# Autodesk Inventor assembly: roller
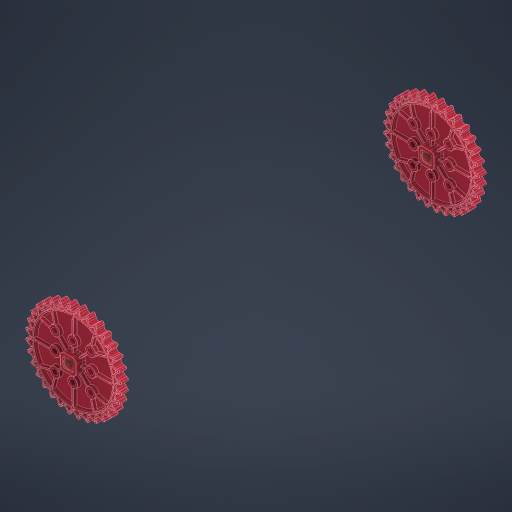
[picture p0: Inventor's stored thumbnail of the model, 512x512]
Saved by Autodesk Inventor 2024 (Build 280153000, 153)
## iProperties
Created: 2023-10-22
Part Number: roller
Document SubType Name: Assembly
Designer: Averey Ku
Author: Averey Ku
## Documents named in this file (3)
- D:\vex_robotics\hardware\cad\spades_v0.1\intake\roller.iam
- D:\vex_robotics\hardware\cad\VEX-CAD-Inventor-1.41\Motion\Sprockets\6P Sprocket.iam
- D:\vex_robotics\hardware\cad\VEX-CAD-Inventor-1.41\Motion\Sprockets\6P Sprocket\6P 32T Sprocket, No Insert.iam
## Components (2 placed, 1 different names)
1. 6P 32T Sprocket, No Insert:3 [sub-assembly] — Insert:2
2. 6P 32T Sprocket, No Insert:4 [sub-assembly] — Insert:2
## Relationships (1: Insert 1)
- Insert:2 (241.3 mm): 6P 32T Sprocket, No Insert:3 ↔ 6P 32T Sprocket, No Insert:4
